# Autodesk Inventor assembly: Assembly1
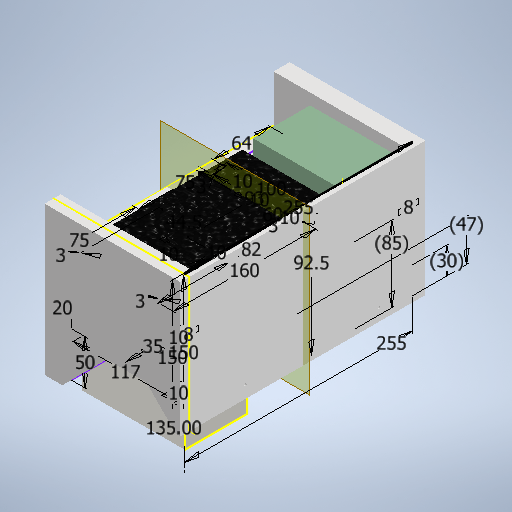
[picture p0: Inventor's stored thumbnail of the model, 512x512]
Saved by Autodesk Inventor 2025.1 (Build 291241000, 241)
## iProperties
Created: 2025-02-21
Part Number: Assembly1
Document SubType Name: Assembly
Designer: m_kni
Author: m_kni
## Documents named in this file (6)
- C:\Users\m_kni\OneDrive\Documents\GitHub\Perovskite-Automated-Synthesis-System\CAD\Ebox\Assembly1.iam
- C:\Users\m_kni\OneDrive\Documents\GitHub\Perovskite-Automated-Synthesis-System\CAD\PSU.ipt
- C:\Users\m_kni\OneDrive\Documents\GitHub\Perovskite-Automated-Synthesis-System\CAD\Spectro.ipt
- C:\Users\m_kni\OneDrive\Documents\GitHub\Perovskite-Automated-Synthesis-System\CAD\Octopus_Board.ipt
- C:\Users\m_kni\OneDrive\Documents\GitHub\Perovskite-Automated-Synthesis-System\CAD\RasPi.ipt
- C:\Users\m_kni\OneDrive\Documents\GitHub\Perovskite-Automated-Synthesis-System\CAD\EboxCase.ipt
## Components (5 placed, 5 different names)
1. PSU:1 — Flush:1, Mate:1, Flush:2, Flush:3, Flush:6, Mate:4, Mate:5, Flush:7
2. Spectro:1 — Flush:1, Mate:1, Flush:2, Mate:2
3. Octopus_Board:1 — Mate:2, Mate:3, Flush:3, Flush:4, Flush:5, Flush:6
4. RasPi:1 — Mate:3, Flush:4, Flush:5
5. EboxCase:1 — Mate:4, Mate:5, Flush:7
## Relationships (12: Flush 7, Mate 5)
- Flush:1: PSU:1 ↔ Spectro:1
- Mate:1 (15 mm): PSU:1 ↔ Spectro:1
- Flush:2 (60 mm): PSU:1 ↔ Spectro:1
- Mate:2 (15 mm): Spectro:1 ↔ Octopus_Board:1
- Mate:3 (5 mm): Octopus_Board:1 ↔ RasPi:1
- Flush:3 (7.5 mm): PSU:1 ↔ Octopus_Board:1
- Flush:4: Octopus_Board:1 ↔ RasPi:1
- Flush:5: Octopus_Board:1 ↔ RasPi:1
- Flush:6 (-12 mm): PSU:1 ↔ Octopus_Board:1
- Mate:4: PSU:1 ↔ EboxCase:1
- Mate:5: PSU:1 ↔ EboxCase:1
- Flush:7: PSU:1 ↔ EboxCase:1
